# Autodesk Inventor assembly: Live Axle Assembly
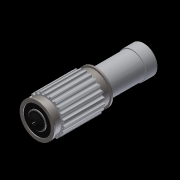
[picture p0: Inventor's stored thumbnail of the model, 180x180]
Saved by Autodesk Inventor 2014 SP1 (Build 180222100, 222)
## iProperties
Created: 2013-11-29
Part Number: Live Axle Assembly
Document SubType Name: Assembly
Designer: Rauhul Varma
Author: Rauhul Varma
## Documents named in this file (7)
- C:\Users\Rauhul Varma\Desktop\2014 Base\Live Axle Assembly.iam
- C:\Users\Rauhul Varma\Desktop\2014 Base\Live Axle.ipt
- C:\Users\Rauhul Varma\Desktop\2014 Base\FBHCS .25-20 .5000 Long.ipt
- C:\Users\Rauhul Varma\Desktop\2014 Base\FR8-2RS Bearing.ipt
- C:\Users\Rauhul Varma\Desktop\2014 Base\22T 5mm GT2 Pulley.ipt
- C:\Users\Rauhul Varma\Desktop\2014 Base\3.5 in by 1.25 in Colson Wheel.ipt
- C:\Users\Rauhul Varma\Desktop\2014 Base\Colson Hub.ipt
## Components (8 placed, 6 different names)
1. Live Axle:1 — Mate:1, Mate:2, Mate:3, Mate:4, Mate:5, Mate:6, Mate:7, Mate:8, Mate:9, Mate:10, Mate:13, Mate:14
2. FBHCS .25-20 .5000 Long:1 — Mate:1, Mate:4
3. FBHCS .25-20 .5000 Long:2 — Mate:2, Mate:3
4. FR8-2RS Bearing:1 — Mate:5, Mate:8, Mate:11, Mate:15
5. FR8-2RS Bearing:2 — Mate:6, Mate:7
6. 22T 5mm GT2 Pulley:1 — Mate:9, Mate:10, Mate:11
7. 3.5 in by 1.25 in Colson Wheel:1 — Mate:12, Mate:13, Mate:16
8. Colson Hub:1 — Mate:12, Mate:14, Mate:15, Mate:16
## Relationships (16: Mate 16)
- Mate:1: Live Axle:1 ↔ FBHCS .25-20 .5000 Long:1
- Mate:2: Live Axle:1 ↔ FBHCS .25-20 .5000 Long:2
- Mate:3: Live Axle:1 ↔ FBHCS .25-20 .5000 Long:2
- Mate:4: Live Axle:1 ↔ FBHCS .25-20 .5000 Long:1
- Mate:5: Live Axle:1 ↔ FR8-2RS Bearing:1
- Mate:6: Live Axle:1 ↔ FR8-2RS Bearing:2
- Mate:7: Live Axle:1 ↔ FR8-2RS Bearing:2
- Mate:8: Live Axle:1 ↔ FR8-2RS Bearing:1
- Mate:9: Live Axle:1 ↔ 22T 5mm GT2 Pulley:1
- Mate:10: Live Axle:1 ↔ 22T 5mm GT2 Pulley:1
- Mate:11: FR8-2RS Bearing:1 ↔ 22T 5mm GT2 Pulley:1
- Mate:12: 3.5 in by 1.25 in Colson Wheel:1 ↔ Colson Hub:1
- Mate:13: Live Axle:1 ↔ 3.5 in by 1.25 in Colson Wheel:1
- Mate:14: Live Axle:1 ↔ Colson Hub:1
- Mate:15: FR8-2RS Bearing:1 ↔ Colson Hub:1
- Mate:16: 3.5 in by 1.25 in Colson Wheel:1 ↔ Colson Hub:1
